# Autodesk Inventor assembly: center_2p_female
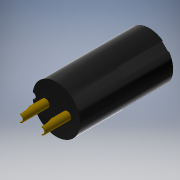
[picture p0: Inventor's stored thumbnail of the model, 180x180]
Saved by Autodesk Inventor 2018 (Build 220112000, 112)
## iProperties
Created: 2019-04-17
Part Number: center_2p_female
Document SubType Name: Assembly
Designer: ZEUSLAP
Author: ZEUSLAP
## Documents named in this file (3)
- C:\Users\Vadim\Desktop\sp16-waterproof-connector-1.snapshot.3\parts\center_2p_female.iam
- C:\Users\Vadim\Desktop\sp16-waterproof-connector-1.snapshot.3\parts\center_2p_female_body.ipt
- C:\Users\Vadim\Desktop\sp16-waterproof-connector-1.snapshot.3\parts\pin_1.8mm.ipt
## Components (3 placed, 2 different names)
1. center_2p_female_body:1 — Angle:1, Angle:2, Mate:1, Angle:3, Mate:2, Angle:4, Flush:2
2. pin_1.8mm:1 — Angle:3, Mate:2, Flush:1, Angle:5, Flush:2
3. pin_1.8mm:2 — Angle:2, Mate:1, Flush:1, Angle:6
## Relationships (10: Angle 6, Mate 2, Flush 2)
- Angle:1 (0 deg): center_2p_female_body:1
- Angle:2 (0 deg): center_2p_female_body:1 ↔ pin_1.8mm:2
- Mate:1: center_2p_female_body:1 ↔ pin_1.8mm:2
- Angle:3 (0 deg): center_2p_female_body:1 ↔ pin_1.8mm:1
- Mate:2: center_2p_female_body:1 ↔ pin_1.8mm:1
- Flush:1: pin_1.8mm:1 ↔ pin_1.8mm:2
- Angle:4 (180 deg): center_2p_female_body:1
- Angle:5 (90 deg): pin_1.8mm:1
- Angle:6 (90 deg): pin_1.8mm:2
- Flush:2 (6 mm): center_2p_female_body:1 ↔ pin_1.8mm:1
